# Autodesk Inventor assembly: HUDSON-1-89
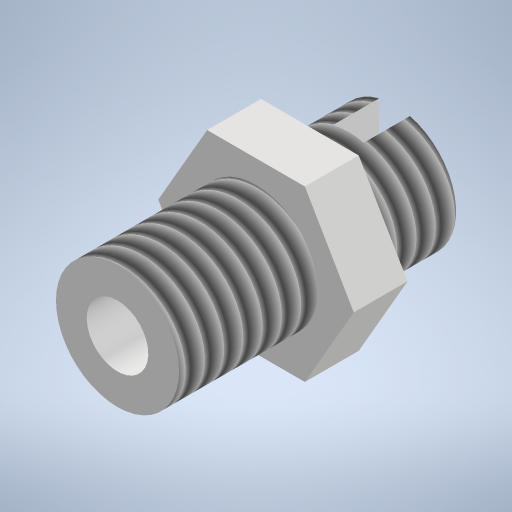
[picture p0: Inventor's stored thumbnail of the model, 512x512]
Saved by Autodesk Inventor 2024.2 (Build 282272000, 272)
## iProperties
Created: 2024-10-06
Part Number: HUDSON-1-89
Document SubType Name: Assembly
Designer: melim
Author: melim
## Documents named in this file (3)
- C:\Users\melim\OneDrive\Desktop\PIEZAS_MELISSA\HUDSON-1-89.iam
- C:\Users\melim\OneDrive\Desktop\PIEZAS_MELISSA\HUDSON-1-89A.ipt
- C:\Users\melim\OneDrive\Desktop\PIEZAS_MELISSA\HUDSON-1-89B.ipt
## Components (2 placed, 2 different names)
1. HUDSON-1-89A:1 — Mate:1, Mate:2
2. HUDSON-1-89B:1 — Mate:1, Mate:2
## Relationships (2: Mate 2)
- Mate:1: HUDSON-1-89A:1 ↔ HUDSON-1-89B:1
- Mate:2 (9 mm): HUDSON-1-89A:1 ↔ HUDSON-1-89B:1
